# Autodesk Inventor assembly: FrontTube
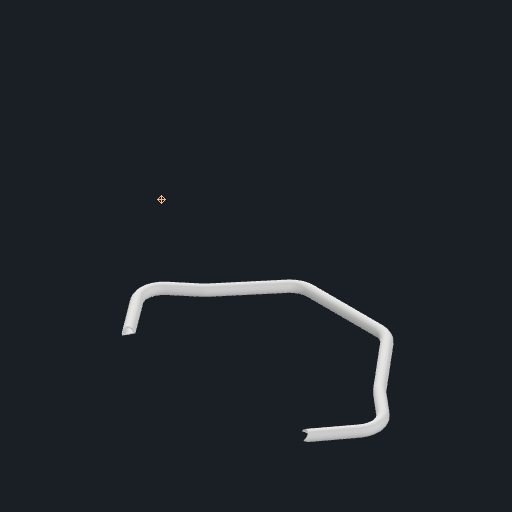
[picture p0: Inventor's stored thumbnail of the model, 512x512]
Saved by Autodesk Inventor 2025.2 (Build 292293000, 293)
## iProperties
Created: 2025-04-01
Part Number: FrontTube
Document SubType Name: Assembly
Designer: valer
Author: valer
## Documents named in this file (2)
- C:\Users\valer\Desktop\str1ker\cad\FrontTube.iam
- C:\Users\valer\Desktop\str1ker\cad\ChestFrontTube.ipt
## Components (1 placed, 1 different names)
1. ChestFrontTube:1 — Angle:1, Mate:1, Mate:2
## Relationships (3: Mate 2, Angle 1)
- Angle:1 (90 deg): ChestFrontTube:1
- Mate:1: ChestFrontTube:1
- Mate:2: ChestFrontTube:1
